# Autodesk Inventor assembly: Level Gauge Assembly
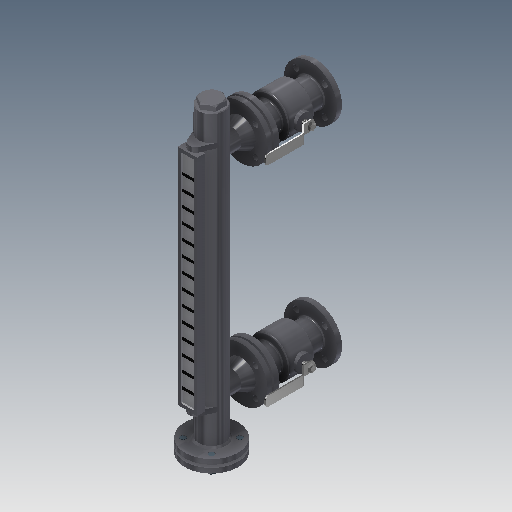
[picture p0: Inventor's stored thumbnail of the model, 512x512]
Saved by Autodesk Inventor 2020 (Build 240152000, 152)
## iProperties
Created: 2009-08-10
Part Number: Level Gauge Assembly
Document SubType Name: Assembly
Designer: Demir Ali
Description: Level Gauge Assembly
Stock Number: NA
Author: Demir Ali
Title: In House Assembly
Revision Number: A
## Documents named in this file (3)
- C:\Users\hallc\Desktop\Process Equipment\Workspace\Options\Level Gauge Assembly.iam
- C:\Users\hallc\Desktop\Process Equipment\Workspace\Options\Bypass Level Gauge.ipt
- C:\Users\hallc\Desktop\Process Equipment\Workspace\Supplier Content\Valves\Flanged Ball Valve - 50NB PN16.iam
## Components (3 placed, 2 different names)
1. Bypass Level Gauge — Insert:1, Insert:2, Mate:1, Mate:2
2. Flanged Ball Valve - 50NB PN16:1 [sub-assembly] — Insert:1, Mate:1
3. Flanged Ball Valve - 50NB PN16:2 [sub-assembly] — Insert:2, Mate:2
## Relationships (4: Insert 2, Mate 2)
- Insert:1: Bypass Level Gauge ↔ Flanged Ball Valve - 50NB PN16:1
- Insert:2: Bypass Level Gauge ↔ Flanged Ball Valve - 50NB PN16:2
- Mate:1: Bypass Level Gauge ↔ Flanged Ball Valve - 50NB PN16:1
- Mate:2: Bypass Level Gauge ↔ Flanged Ball Valve - 50NB PN16:2
